# Autodesk Inventor assembly: wheel
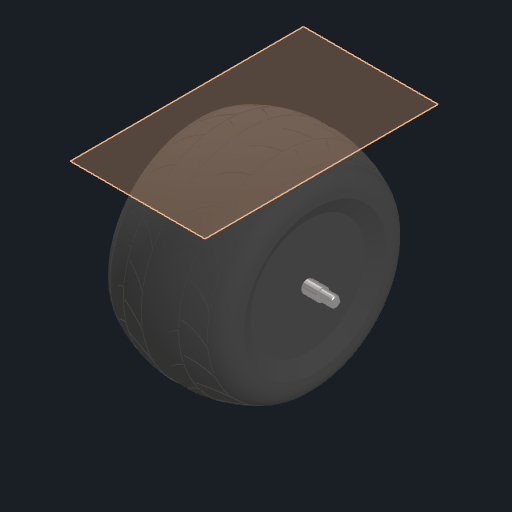
[picture p0: Inventor's stored thumbnail of the model, 512x512]
Saved by Autodesk Inventor 2024 (Build 280153000, 153)
## iProperties
Created: 2024-04-30
Part Number: wheel
Document SubType Name: Assembly
Designer: markm
Author: markm
## Documents named in this file (3)
- C:\Users\markm\OneDrive\Документы\Inventor\eventide\wheel\wheel.iam
- C:\Users\markm\OneDrive\Документы\Inventor\eventide\wheel\tire.ipt
- C:\Users\markm\OneDrive\Документы\Inventor\eventide\wheel\axel.ipt
## Components (2 placed, 2 different names)
1. tire:1
2. axel:1 — Mate:1, Flush:1
## Relationships (2: Mate 1, Flush 1)
- Mate:1: axel:1
- Flush:1: axel:1
